# Autodesk Inventor assembly: Assembly1
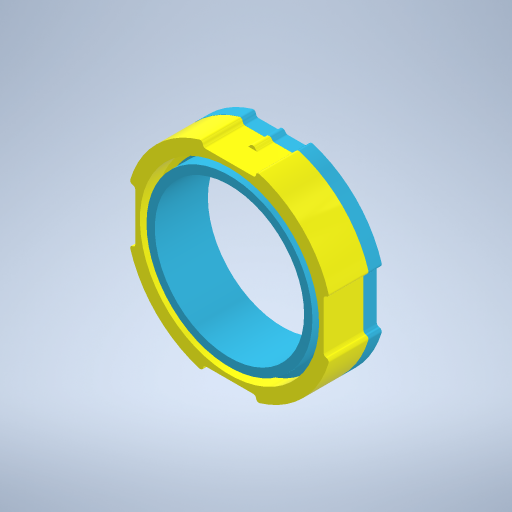
[picture p0: Inventor's stored thumbnail of the model, 512x512]
Saved by Autodesk Inventor 2023.2 (Build 272271030, 271C)
## iProperties
Created: 2023-10-23
Part Number: Assembly1
Document SubType Name: Assembly
Designer: Cris Pat
Author: Cris Pat
## Documents named in this file (5)
- C:\Users\Cris Pat\Desktop\U\Semestre_10\Disenio_y_manufactura\proyecto2\Assembly1.iam
- C:\Users\Cris Pat\Desktop\U\Semestre_10\Disenio_y_manufactura\proyecto2\rosca_1.ipt
- C:\Users\Cris Pat\Desktop\U\Semestre_10\Disenio_y_manufactura\proyecto2\rosca_2.ipt
- C:\Users\Cris Pat\Desktop\U\Semestre_10\Disenio_y_manufactura\proyecto2\Assembly1\Design Accelerator\Tolerance1.iam
- C:\Users\Cris Pat\Desktop\U\Semestre_10\Disenio_y_manufactura\proyecto2\Assembly1\Design Accelerator\Tolerance2.iam
## Components (4 placed, 3 different names)
1. rosca_1:1 — Rotational:1, Rotational:2
2. rosca_2:1 — Rotational:1, Rotational:2
3. Tolerance:1 [sub-assembly]
4. Tolerance:2 [sub-assembly]
## Relationships (2: RevoluteJoint 2)
- Rotational:1 [RevoluteJoint]: rosca_1:1 ↔ rosca_2:1
- Rotational:2 [RevoluteJoint]: rosca_1:1 ↔ rosca_2:1
